# Autodesk Inventor assembly: 部件3
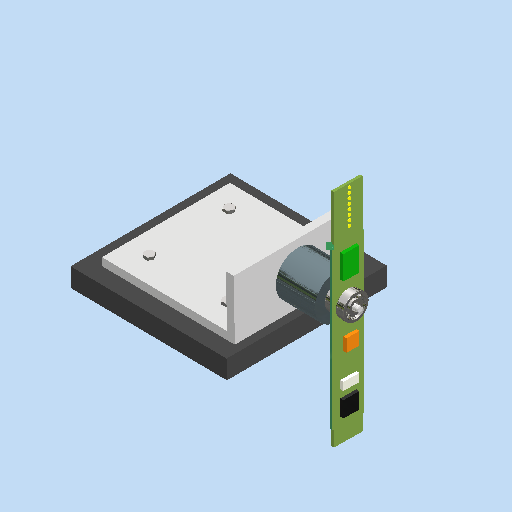
[picture p0: Inventor's stored thumbnail of the model, 512x512]
Saved by Autodesk Inventor 2026.2 (Build 302298010, 298A)
## iProperties
Created: 2026-03-16
Part Number: 部件3
Document SubType Name: Assembly
Designer: liu
Author: liu
## Documents named in this file (9)
- C:\Users\25710\Desktop\旋转LED建模\部件3.iam
- C:\Users\25710\Desktop\旋转LED建模\pcb板.ipt
- C:\Users\25710\Desktop\旋转LED建模\底座.ipt
- C:\Users\25710\Desktop\旋转LED建模\电机.ipt
- C:\Users\25710\Desktop\旋转LED建模\电机底座.ipt
- C:\Users\25710\Documents\Inventor\Content Center Files\R2026\zh-CN\GB_T 5782-2000\螺栓 GB_T 5782 M3 x 20.ipt
- C:\Users\25710\Documents\Inventor\Content Center Files\R2026\zh-CN\GB_T 6170-2000\螺母 GB_T 6170 M3.ipt
- C:\Users\25710\Documents\Inventor\Content Center Files\R2026\zh-CN\GB_T 276-94 60000-2RS and 2LS\轴承 625-2LS GB_T 276-94.ipt
- C:\Users\25710\Documents\Inventor\Content Center Files\R2026\zh-CN\GB 809-88 A\螺母 GB 809 A M3 x 3.ipt
## Components (15 placed, 8 different names)
1. pcb板:1 — 配合:4, 配合:19
2. 底座:1 — 配合:1, 配合:2, 配合:6, 配合:7, 配合:9, 配合:10, 配合:11, 配合:13, 配合:15
3. 电机:1 — 配合:3, 表面齐平:1, 配合:4, 配合:16, 配合:17, 配合:18, 配合:20
4. 电机底座:1 — 配合:1, 配合:2, 配合:3, 表面齐平:1, 插入:3, 插入:4, 插入:5, 插入:6
5. 螺栓 GB/T 5782-2000 M3x20:3 — 插入:3, 配合:5
6. 螺母 GB/T 6170-2000 M3:1 — 配合:5, 配合:6
7. 螺栓 GB/T 5782-2000 M3x20:4 — 插入:4, 配合:7, 配合:8
8. 螺母 GB/T 6170-2000 M3:2 — 配合:8, 配合:9
9. 螺栓 GB/T 5782-2000 M3x20:5 — 插入:5, 配合:10, 配合:14
10. 螺栓 GB/T 5782-2000 M3x20:6 — 插入:6, 配合:11, 配合:12
11. 螺母 GB/T 6170-2000 M3:3 — 配合:12, 配合:13
12. 螺母 GB/T 6170-2000 M3:4 — 配合:14, 配合:15
13. 滚动轴承 GB/T 276-1994 60000-2RS 和 2LS 型 625-2LS:1 — 配合:16, 配合:17
14. 滚动轴承 GB/T 276-1994 60000-2RS 和 2LS 型 625-2LS:2 — 配合:18, 配合:19, 插入:7
15. 螺母 GB/T 809-1988 A 型 M3x3:1 — 插入:7, 配合:20
## Relationships (26: Mate 20, Insert 5, Flush 1)
- 配合:1 [Mate]: 底座:1 ↔ 电机底座:1
- 配合:2 [Mate] (5 mm): 底座:1 ↔ 电机底座:1
- 配合:3 [Mate]: 电机:1 ↔ 电机底座:1
- 表面齐平:1 [Flush]: 电机:1 ↔ 电机底座:1
- 配合:4 [Mate]: pcb板:1 ↔ 电机:1
- 插入:3 [Insert]: 电机底座:1 ↔ 螺栓 GB/T 5782-2000 M3x20:3
- 配合:5 [Mate]: 螺栓 GB/T 5782-2000 M3x20:3 ↔ 螺母 GB/T 6170-2000 M3:1
- 配合:6 [Mate]: 底座:1 ↔ 螺母 GB/T 6170-2000 M3:1
- 插入:4 [Insert]: 电机底座:1 ↔ 螺栓 GB/T 5782-2000 M3x20:4
- 配合:7 [Mate]: 底座:1 ↔ 螺栓 GB/T 5782-2000 M3x20:4
- 配合:8 [Mate]: 螺栓 GB/T 5782-2000 M3x20:4 ↔ 螺母 GB/T 6170-2000 M3:2
- 配合:9 [Mate]: 底座:1 ↔ 螺母 GB/T 6170-2000 M3:2
- 插入:5 [Insert]: 电机底座:1 ↔ 螺栓 GB/T 5782-2000 M3x20:5
- 配合:10 [Mate]: 底座:1 ↔ 螺栓 GB/T 5782-2000 M3x20:5
- 插入:6 [Insert]: 电机底座:1 ↔ 螺栓 GB/T 5782-2000 M3x20:6
- 配合:11 [Mate]: 底座:1 ↔ 螺栓 GB/T 5782-2000 M3x20:6
- 配合:12 [Mate]: 螺栓 GB/T 5782-2000 M3x20:6 ↔ 螺母 GB/T 6170-2000 M3:3
- 配合:13 [Mate]: 底座:1 ↔ 螺母 GB/T 6170-2000 M3:3
- 配合:14 [Mate]: 螺栓 GB/T 5782-2000 M3x20:5 ↔ 螺母 GB/T 6170-2000 M3:4
- 配合:15 [Mate]: 底座:1 ↔ 螺母 GB/T 6170-2000 M3:4
- 配合:16 [Mate]: 电机:1 ↔ 滚动轴承 GB/T 276-1994 60000-2RS 和 2LS 型 625-2LS:1
- 配合:17 [Mate]: 电机:1 ↔ 滚动轴承 GB/T 276-1994 60000-2RS 和 2LS 型 625-2LS:1
- 配合:18 [Mate]: 电机:1 ↔ 滚动轴承 GB/T 276-1994 60000-2RS 和 2LS 型 625-2LS:2
- 配合:19 [Mate]: pcb板:1 ↔ 滚动轴承 GB/T 276-1994 60000-2RS 和 2LS 型 625-2LS:2
- 插入:7 [Insert]: 滚动轴承 GB/T 276-1994 60000-2RS 和 2LS 型 625-2LS:2 ↔ 螺母 GB/T 809-1988 A 型 M3x3:1
- 配合:20 [Mate]: 电机:1 ↔ 螺母 GB/T 809-1988 A 型 M3x3:1
